# Autodesk Inventor assembly: TempLoggerBox-v2
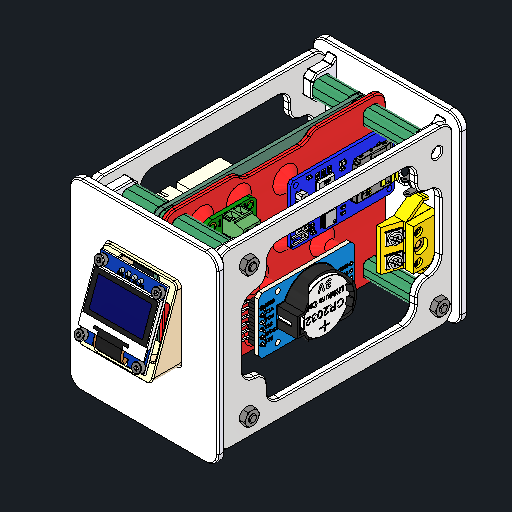
[picture p0: Inventor's stored thumbnail of the model, 512x512]
Saved by Autodesk Inventor 2027.1 (Build 311270010, 270A)
## iProperties
Created: 2025-07-16
Part Number: TempLoggerBox-v2
Document SubType Name: Assembly
Designer: kuzmin
Author: kuzmin
## Documents named in this file (21)
- C:\Users\queezz\Dropbox\Drawings\pihti-cad\ElectronicsBox\esp32-ambient-logger\TempLoggerBox-v2.iam
- C:\Users\queezz\Dropbox\Drawings\pihti-cad\ElectronicsBox\esp32-ambient-logger\TempLoggerRev1.iam
- C:\Users\queezz\Dropbox\Drawings\pihti-cad\ElectronicsBox\esp32-ambient-logger\STEPs\ESP32-DevkitC32U.iam
- C:\Users\queezz\Dropbox\Drawings\pihti-cad\ElectronicsBox\esp32-ambient-logger\STEPs\DS3231 RTC\DS2321 RTC.ipt
- C:\Users\queezz\Dropbox\Drawings\pihti-cad\ElectronicsBox\esp32-ambient-logger\STEPs\OLED-128x64-0.96.ipt
- C:\Users\queezz\Dropbox\Drawings\pihti-cad\ElectronicsBox\esp32-ambient-logger\STEPs\Product_TF Micro SD Card Memory Modul .iam
- C:\Users\queezz\Dropbox\Drawings\pihti-cad\ElectronicsBox\TempController-v2\STEPs\Type-K Thermocouple Mini Socket\Type-K Thermocouple Mini Socket.iam
- C:\Users\queezz\Dropbox\Drawings\pihti-cad\ContentCenter\Electrics\DC Jack Panel Mount Base.ipt
- C:\Users\queezz\Dropbox\Drawings\pihti-cad\ElectronicsBox\esp32-ambient-logger\STEPs\Adafruit_MAX31855.iam
- C:\Users\queezz\Dropbox\Drawings\pihti-cad\ElectronicsBox\esp32-ambient-logger\temp-logger-shelf-v2.ipt
- C:\Users\queezz\Dropbox\Drawings\pihti-cad\ElectronicsBox\esp32-ambient-logger\shaft-10mm.ipt
- C:\Users\queezz\Dropbox\Drawings\pihti-cad\ElectronicsBox\esp32-ambient-logger\shaft-20mm-squareipt.ipt
- C:\Users\queezz\Dropbox\Drawings\pihti-cad\ElectronicsBox\esp32-ambient-logger\temp-logger-base-plate-v2.ipt
- C:\Users\queezz\Dropbox\Drawings\pihti-cad\ElectronicsBox\esp32-ambient-logger\shaft-15mm-squareipt.ipt
- C:\Users\queezz\Dropbox\Drawings\pihti-cad\ElectronicsBox\esp32-ambient-logger\temp-logger-back-plate-v2.ipt
- C:\Users\queezz\Dropbox\Drawings\pihti-cad\ContentCenter\Fastners\M3-nut.ipt
- C:\Users\queezz\Dropbox\Drawings\pihti-cad\ElectronicsBox\esp32-ambient-logger\temp-logger-front-plate-v2.ipt
- C:\Users\queezz\Dropbox\Drawings\pihti-cad\ElectronicsBox\esp32-ambient-logger\m3-60-pin.ipt
- C:\Users\queezz\Dropbox\Drawings\pihti-cad\ElectronicsBox\esp32-ambient-logger\oled-screen-mount.ipt
- C:\Users\queezz\Dropbox\Drawings\pihti-cad\ContentCenter\Fastners\M2x4-SHCS.ipt
- C:\Users\queezz\Dropbox\Drawings\pihti-cad\ElectronicsBox\esp32-ambient-logger\enclosure.ipt
## Components (43 placed, 20 different names)
1. TempLoggerRev1:1 [sub-assembly] — Mate:1, Flush:1, Flush:2, Rigid:1, Rigid:2, Rigid:3, Rigid:4, Rigid:11, Rigid:12, Rigid:13, Rigid:14
2. ESP32-DevkitC32U:1 [sub-assembly] — Mate:1, Flush:1, Flush:2
3. DS2321 RTC:1 — Mate:5, Mate:6, Mate:7
4. OLED-128x64-0.96:1 — Rigid:39, Rigid:40, Rigid:41, Rigid:42, Rigid:43
5. Product_TF Micro SD Card Memory Modul :1 [sub-assembly] — Mate:2, Mate:3, Mate:4
6. Type-K Thermocouple Mini Socket:1 [sub-assembly] — Mate:20, Mate:21, Mate:22
7. DC Jack Panel Mount Base:1 — Rotational:2
8. Adafruit_MAX31855:1 [sub-assembly] — Mate:8, Mate:9, Mate:10
9. temp-logger-shelf-v2:1 — Rigid:5, Mate:2, Mate:3, Mate:4, Mate:5, Mate:6, Rigid:6, Rigid:7, Rigid:8, Rigid:9, Mate:7, Mate:8, Mate:9, Mate:10
10. shaft-10mm:1 — Rigid:2
11. shaft-10mm:2 — Rigid:1, Rigid:5
12. shaft-10mm:3 — Rigid:3
13. shaft-10mm:4 — Rigid:4
14. shaft-20mm-squareipt:1 — Rigid:6, Rigid:25
15. shaft-20mm-squareipt:2 — Rigid:7
16. shaft-20mm-squareipt:3 — Rigid:8
17. shaft-20mm-squareipt:4 — Rigid:9
18. temp-logger-base-plate-v2:1 — Mate:13, Mate:14, Symmetry:1, Mate:15, Flush:3, Rigid:35, Rigid:36, Rigid:37, Rigid:38, Rigid:44
19. temp-logger-base-plate-v2:2 — Symmetry:1, Rigid:31, Rigid:32, Rigid:33, Rigid:34, Rigid:44
20. shaft-15mm-squareipt:1 — Rigid:13
21. shaft-15mm-squareipt:2 — Rigid:12
22. shaft-15mm-squareipt:3 — Rigid:11
23. shaft-15mm-squareipt:4 — Rigid:14
24. temp-logger-back-plate-v2:1 — Mate:13, Mate:17, Flush:4, Rigid:25, Mate:20, Mate:21, Mate:22, Rotational:2, Mate:28
25. temp-logger-front-plate-v2:1 — Mate:14, Mate:18, Mate:19, Mate:23, Mate:24, Mate:25
26. m3-60-pin:1 — Rigid:27
27. m3-60-pin:2 — Rigid:28
28. m3-60-pin:3 — Rigid:30
29. m3-60-pin:4 — Rigid:29
30. oled-screen-mount:1 — Mate:23, Mate:24, Mate:25, Rigid:43
31. enclosure:1 — Mate:26, Mate:27, Mate:28
32. SS ISO 4762 M2 x 4:1 — Rigid:39
33. SS ISO 4762 M2 x 4:2 — Rigid:40
34. SS ISO 4762 M2 x 4:3 — Rigid:41
35. SS ISO 4762 M2 x 4:4 — Rigid:42
36. JIS B 1181 Style 1 - Metric A M3:1 — Rigid:29, Rigid:37
37. JIS B 1181 Style 1 - Metric A M3:2 — Rigid:33
38. JIS B 1181 Style 1 - Metric A M3:3 — Rigid:32
39. JIS B 1181 Style 1 - Metric A M3:4 — Rigid:30, Rigid:35
40. JIS B 1181 Style 1 - Metric A M3:5 — Rigid:27, Rigid:36
41. JIS B 1181 Style 1 - Metric A M3:6 — Rigid:31
42. JIS B 1181 Style 1 - Metric A M3:7 — Rigid:34
43. JIS B 1181 Style 1 - Metric A M3:8 — Rigid:28, Rigid:38
## Relationships (64: WeldJoint 32, Mate 26, Flush 4, Symmetry 1, RevoluteJoint 1)
- Mate:1: TempLoggerRev1:1 ↔ ESP32-DevkitC32U:1
- Flush:1: TempLoggerRev1:1 ↔ ESP32-DevkitC32U:1
- Flush:2: TempLoggerRev1:1 ↔ ESP32-DevkitC32U:1
- Rigid:1 [WeldJoint]: TempLoggerRev1:1 ↔ shaft-10mm:2
- Rigid:2 [WeldJoint]: TempLoggerRev1:1 ↔ shaft-10mm:1
- Rigid:3 [WeldJoint]: TempLoggerRev1:1 ↔ shaft-10mm:3
- Rigid:4 [WeldJoint]: TempLoggerRev1:1 ↔ shaft-10mm:4
- Rigid:5 [WeldJoint]: temp-logger-shelf-v2:1 ↔ shaft-10mm:2
- Mate:2: Product_TF Micro SD Card Memory Modul :1 ↔ temp-logger-shelf-v2:1
- Mate:3: Product_TF Micro SD Card Memory Modul :1 ↔ temp-logger-shelf-v2:1
- Mate:4: Product_TF Micro SD Card Memory Modul :1 ↔ temp-logger-shelf-v2:1
- Mate:5: DS2321 RTC:1 ↔ temp-logger-shelf-v2:1
- Mate:6: DS2321 RTC:1 ↔ temp-logger-shelf-v2:1
- Rigid:6 [WeldJoint]: temp-logger-shelf-v2:1 ↔ shaft-20mm-squareipt:1
- Rigid:7 [WeldJoint]: temp-logger-shelf-v2:1 ↔ shaft-20mm-squareipt:2
- Rigid:8 [WeldJoint]: temp-logger-shelf-v2:1 ↔ shaft-20mm-squareipt:3
- Rigid:9 [WeldJoint]: temp-logger-shelf-v2:1 ↔ shaft-20mm-squareipt:4
- Mate:7: DS2321 RTC:1 ↔ temp-logger-shelf-v2:1
- Mate:8: Adafruit_MAX31855:1 ↔ temp-logger-shelf-v2:1
- Mate:9: Adafruit_MAX31855:1 ↔ temp-logger-shelf-v2:1
- Mate:10: Adafruit_MAX31855:1 ↔ temp-logger-shelf-v2:1
- Rigid:11 [WeldJoint]: TempLoggerRev1:1 ↔ shaft-15mm-squareipt:3
- Rigid:12 [WeldJoint]: TempLoggerRev1:1 ↔ shaft-15mm-squareipt:2
- Rigid:13 [WeldJoint]: TempLoggerRev1:1 ↔ shaft-15mm-squareipt:1
- Rigid:14 [WeldJoint]: TempLoggerRev1:1 ↔ shaft-15mm-squareipt:4
- Mate:13: temp-logger-base-plate-v2:1 ↔ temp-logger-back-plate-v2:1
- Mate:14: temp-logger-base-plate-v2:1 ↔ temp-logger-front-plate-v2:1
- Symmetry:1: temp-logger-base-plate-v2:1 ↔ temp-logger-base-plate-v2:2
- Mate:15: temp-logger-base-plate-v2:1
- Mate:16
- Flush:3: temp-logger-base-plate-v2:1
- Mate:17: temp-logger-back-plate-v2:1
- Flush:4: temp-logger-back-plate-v2:1
- Mate:18: temp-logger-front-plate-v2:1
- Mate:19: temp-logger-front-plate-v2:1
- Rigid:25 [WeldJoint]: shaft-20mm-squareipt:1 ↔ temp-logger-back-plate-v2:1
- Rigid:27 [WeldJoint] (0.5 mm): m3-60-pin:1 ↔ JIS B 1181 Style 1 - Metric A M3:5
- Rigid:28 [WeldJoint] (0.5 mm): m3-60-pin:2 ↔ JIS B 1181 Style 1 - Metric A M3:8
- Rigid:29 [WeldJoint] (0.5 mm): m3-60-pin:4 ↔ JIS B 1181 Style 1 - Metric A M3:1
- Rigid:30 [WeldJoint] (0.5 mm): m3-60-pin:3 ↔ JIS B 1181 Style 1 - Metric A M3:4
- Mate:20: Type-K Thermocouple Mini Socket:1 ↔ temp-logger-back-plate-v2:1
- Mate:21: Type-K Thermocouple Mini Socket:1 ↔ temp-logger-back-plate-v2:1
- Mate:22: Type-K Thermocouple Mini Socket:1 ↔ temp-logger-back-plate-v2:1
- Mate:23: temp-logger-front-plate-v2:1 ↔ oled-screen-mount:1
- Mate:24: temp-logger-front-plate-v2:1 ↔ oled-screen-mount:1
- Mate:25: temp-logger-front-plate-v2:1 ↔ oled-screen-mount:1
- Rigid:31 [WeldJoint]: temp-logger-base-plate-v2:2 ↔ JIS B 1181 Style 1 - Metric A M3:6
- Rigid:32 [WeldJoint]: temp-logger-base-plate-v2:2 ↔ JIS B 1181 Style 1 - Metric A M3:3
- Rigid:33 [WeldJoint]: temp-logger-base-plate-v2:2 ↔ JIS B 1181 Style 1 - Metric A M3:2
- Rigid:34 [WeldJoint]: temp-logger-base-plate-v2:2 ↔ JIS B 1181 Style 1 - Metric A M3:7
- Rigid:35 [WeldJoint]: temp-logger-base-plate-v2:1 ↔ JIS B 1181 Style 1 - Metric A M3:4
- Rigid:36 [WeldJoint]: temp-logger-base-plate-v2:1 ↔ JIS B 1181 Style 1 - Metric A M3:5
- Rigid:37 [WeldJoint]: temp-logger-base-plate-v2:1 ↔ JIS B 1181 Style 1 - Metric A M3:1
- Rigid:38 [WeldJoint]: temp-logger-base-plate-v2:1 ↔ JIS B 1181 Style 1 - Metric A M3:8
- Rigid:39 [WeldJoint]: OLED-128x64-0.96:1 ↔ SS ISO 4762 M2 x 4:1
- Rigid:40 [WeldJoint]: OLED-128x64-0.96:1 ↔ SS ISO 4762 M2 x 4:2
- Rigid:41 [WeldJoint]: OLED-128x64-0.96:1 ↔ SS ISO 4762 M2 x 4:3
- Rigid:42 [WeldJoint]: OLED-128x64-0.96:1 ↔ SS ISO 4762 M2 x 4:4
- Rotational:2 [RevoluteJoint]: DC Jack Panel Mount Base:1 ↔ temp-logger-back-plate-v2:1
- Mate:26: enclosure:1
- Mate:27: enclosure:1
- Mate:28: temp-logger-back-plate-v2:1 ↔ enclosure:1
- Rigid:43 [WeldJoint]: OLED-128x64-0.96:1 ↔ oled-screen-mount:1
- Rigid:44 [WeldJoint] (48 mm): temp-logger-base-plate-v2:1 ↔ temp-logger-base-plate-v2:2
